# Autodesk Inventor assembly: support orangepi
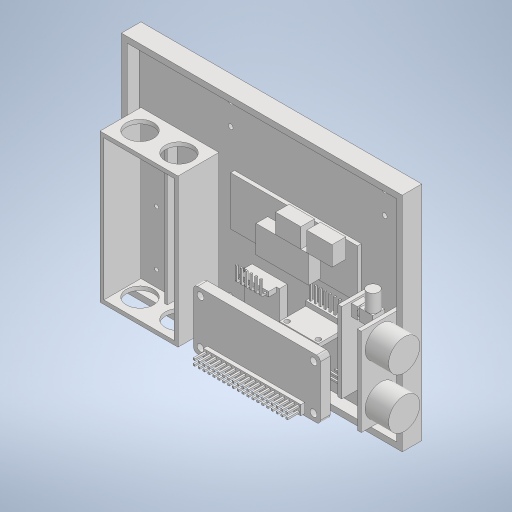
[picture p0: Inventor's stored thumbnail of the model, 512x512]
Saved by Autodesk Inventor 2024 (Build 280153000, 153)
## iProperties
Created: 2024-03-12
Part Number: support orangepi
Document SubType Name: Assembly
Designer: phaly
Author: phaly
## Documents named in this file (10)
- C:\Users\phaly\Music\Perso\Projet voiture\3D\Support\support orangepi.iam
- C:\Users\phaly\Music\Perso\Projet voiture\3D\Support\support.ipt
- C:\Users\phaly\Music\Perso\Projet voiture\3D\Support\couvercle.ipt
- C:\Users\phaly\Music\Perso\Projet voiture\3D\Support\support pile.ipt
- C:\Users\phaly\Music\Perso\Projet voiture\3D\Support\OrangePi.ipt
- C:\Users\phaly\Music\Perso\Projet voiture\3D\Support\Power.ipt
- C:\Users\phaly\Music\Perso\Projet voiture\3D\Support\convertisseur.ipt
- C:\Users\phaly\Music\Perso\Projet voiture\3D\Support\nrf24.ipt
- C:\Users\phaly\Music\Perso\Projet voiture\3D\Support\distance.ipt
- C:\Users\phaly\Music\Perso\Projet voiture\3D\Support\gyro.ipt
## Components (9 placed, 9 different names)
1. support:1 — Placage:1, Affleurement:1, Affleurement:2, Placage:2, Placage:3, Placage:4, Placage:5, Placage:8, Placage:11, Placage:17, Placage:18, Placage:19, Placage:20, Placage:24, Tangente:1, Tangente:2, Placage:25, Placage:28, Placage:29, Placage:30, Placage:31
2. couvercle:1 — Placage:1, Affleurement:1, Affleurement:2
3. support pile:1 — Placage:2, Placage:3, Placage:4
4. OrangePi:1 — Placage:5, Placage:18, Placage:19, Affleurement:3, Affleurement:6
5. Power:1 — Placage:8, Placage:17, Placage:20
6. convertisseur:1 — Placage:11, Placage:25, Affleurement:3, Affleurement:5
7. distance:1 — Placage:24, Tangente:1, Tangente:2
8. nrf24:1 — Placage:29, Placage:30, Placage:31
9. gyro:1 — Placage:28, Affleurement:5, Affleurement:6
## Relationships (24: Mate 17, Flush 5, Tangent 2)
- Placage:1 [Mate]: support:1 ↔ couvercle:1
- Affleurement:1 [Flush]: support:1 ↔ couvercle:1
- Affleurement:2 [Flush]: support:1 ↔ couvercle:1
- Placage:2 [Mate]: support:1 ↔ support pile:1
- Placage:3 [Mate] (1 mm): support:1 ↔ support pile:1
- Placage:4 [Mate] (1 mm): support:1 ↔ support pile:1
- Placage:5 [Mate] (18 mm): support:1 ↔ OrangePi:1
- Placage:8 [Mate]: support:1 ↔ Power:1
- Placage:11 [Mate]: support:1 ↔ convertisseur:1
- Placage:17 [Mate] (35 mm): support:1 ↔ Power:1
- Placage:18 [Mate] (5 mm): support:1 ↔ OrangePi:1
- Placage:19 [Mate] (22 mm): support:1 ↔ OrangePi:1
- Placage:20 [Mate] (24 mm): support:1 ↔ Power:1
- Placage:24 [Mate]: support:1 ↔ distance:1
- Tangente:1: support:1 ↔ distance:1
- Tangente:2: support:1 ↔ distance:1
- Placage:25 [Mate]: support:1 ↔ convertisseur:1
- Affleurement:3 [Flush]: OrangePi:1 ↔ convertisseur:1
- Placage:28 [Mate]: support:1 ↔ gyro:1
- Affleurement:5 [Flush]: convertisseur:1 ↔ gyro:1
- Affleurement:6 [Flush]: OrangePi:1 ↔ gyro:1
- Placage:29 [Mate]: support:1 ↔ nrf24:1
- Placage:30 [Mate] (15 mm): support:1 ↔ nrf24:1
- Placage:31 [Mate] (18 mm): support:1 ↔ nrf24:1
